# Autodesk Inventor assembly: звезда и втулка_MIR_MIR
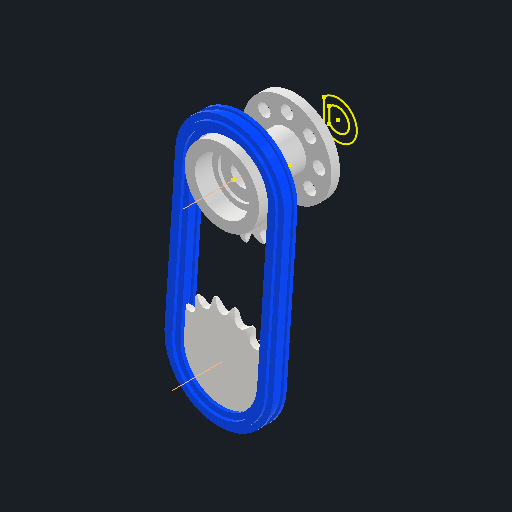
[picture p0: Inventor's stored thumbnail of the model, 512x512]
Saved by Autodesk Inventor 2025 (Build 290162000, 162)
## iProperties
Created: 2024-09-17
Part Number: звезда и втулка_MIR_MIR
Document SubType Name: Assembly
Designer: GameHD
Author: GameHD
## Documents named in this file (3)
- C:\Users\GameHD\Downloads\Telegram Desktop\втулка+подшипники нужная сборка\звезда и втулка_MIR_MIR.iam
- C:\Users\GameHD\Downloads\Telegram Desktop\втулка+подшипники нужная сборка\втулка для подш_MIR_MIR.ipt
- C:\Users\GameHD\Desktop\робототехника\цепь короткая 2.0_MIR_MIR.ipt
## Components (2 placed, 2 different names)
1. втулка для подш_MIR_MIR:1 — Совмещение:1, Заподлицо:1
2. цепь короткая 2.0_MIR_MIR:1 — Совмещение:1, Заподлицо:1
## Relationships (2: Mate 1, Flush 1)
- Совмещение:1 [Mate]: втулка для подш_MIR_MIR:1 ↔ цепь короткая 2.0_MIR_MIR:1
- Заподлицо:1 [Flush] (4 mm): втулка для подш_MIR_MIR:1 ↔ цепь короткая 2.0_MIR_MIR:1
